# Autodesk Inventor assembly: Wago 745-851 (76A) Block
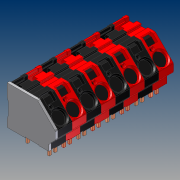
[picture p0: Inventor's stored thumbnail of the model, 180x180]
Saved by Autodesk Inventor 2012 (Build 160160000, 160)
## iProperties
Company: Team 801
Created: 2007-09-01
Part Number: Wago 745-851 (76A) Block
Document SubType Name: Assembly
Designer: Jeffrey M
Catalog Web Link: www.team801.org
Mass: 55.8564 g
Surface Area: 292.703 cm^2
Volume: 55.8564 cm^3
Density: 1 g/cm^3
Author: Jeffrey M
## Documents named in this file (4)
- Z:\UserData\Documents\Inventor\team1885frc\Electronics\PowerDistributionBoard\Wago 745-851 (76A) Block.iam
- Z:\UserData\Documents\Inventor\team1885frc\Electronics\PowerDistributionBoard\Wago 745-500.ipt
- Z:\UserData\Documents\Inventor\team1885frc\Electronics\PowerDistributionBoard\Wago 745-851 (76A) Black.ipt
- Z:\UserData\Documents\Inventor\team1885frc\Electronics\PowerDistributionBoard\Wago 745-851 (76A) Red.ipt
## Components (9 placed, 2 different names)
1. 745-500:1 — Mate:2, Flush:3, Flush:4
2. Wago 745-851 (76A):2 — Mate:1, Flush:1, Flush:2
3. Wago 745-851 (76A):1 — Mate:1, Flush:1, Flush:2, Mate:2, Flush:3, Flush:4
4. Wago 745-851 (76A):3
5. Wago 745-851 (76A):4
6. Wago 745-851 (76A):5
7. Wago 745-851 (76A):6
8. Wago 745-851 (76A):7
9. Wago 745-851 (76A):8
## Component patterns: (4 elements, first: Wago 745-851 (76A):2 + Wago 745-851 (76A):1)
## Relationships (6: Flush 4, Mate 2)
- Mate:1: Wago 745-851 (76A):2 ↔ Wago 745-851 (76A):1
- Flush:1: Wago 745-851 (76A):2 ↔ Wago 745-851 (76A):1
- Flush:2: Wago 745-851 (76A):2 ↔ Wago 745-851 (76A):1
- Mate:2: 745-500:1 ↔ Wago 745-851 (76A):1
- Flush:3: 745-500:1 ↔ Wago 745-851 (76A):1
- Flush:4: 745-500:1 ↔ Wago 745-851 (76A):1
